# Autodesk Inventor assembly: Ball Bearing Inside Mechanics
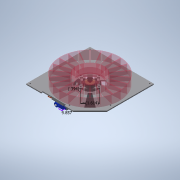
[picture p0: Inventor's stored thumbnail of the model, 180x180]
Saved by Autodesk Inventor 2022 (Build 260153000, 153)
## iProperties
Created: 2023-03-21
Part Number: Ball Bearing Inside Mechanics
Document SubType Name: Assembly
Designer: zarek
Author: zarek
## Documents named in this file (9)
- C:\Users\zarek\OneDrive\Desktop\Random New Stuff\SPB\Ball Bearing Inside Mechanics.iam
- C:\Users\zarek\OneDrive\Desktop\Random New Stuff\SPB\Capsule_Design_Revamp.ipt
- C:\Users\zarek\OneDrive\Desktop\Random New Stuff\SPB\Drop_Plate_Ball_Bearing_Cuttout.ipt
- C:\Users\zarek\OneDrive\Desktop\Random New Stuff\SPB\GrabCad Parts\Stepper 28BYJ48.ipt
- C:\Users\zarek\OneDrive\Desktop\Random New Stuff\SPB\Ball_Bearing_Holder_Assembly.iam
- C:\Users\zarek\OneDrive\Desktop\Random New Stuff\SPB\Ball_Bearing_Mock_8_22_7mm.ipt
- C:\Users\zarek\OneDrive\Desktop\Random New Stuff\SPB\Servo Holder.ipt
- C:\Users\zarek\OneDrive\Desktop\Random New Stuff\SPB\GrabCad Parts\Servo HXT900 Micro.ipt
- C:\Users\zarek\OneDrive\Desktop\Random New Stuff\SPB\Motor_Holder - Copy.ipt
## Components (8 placed, 8 different names)
1. Capsule_Design_Revamp:1 — Rigid:1
2. Stepper 28BYJ48:1 — Rotational:3
3. Ball_Bearing_Holder_Assembly:1 [sub-assembly] — Rotational:3, Rigid:1
4. Drop_Plate_Ball_Bearing_Cuttout:1 — Rigid:2, Rotational:6
5. Ball_Bearing_Mock_8_22_7mm:1
6. Servo Holder:1 — Rigid:2, Rotational:5
7. Servo HXT900 Micro:1 — Rotational:5
8. Motor_Holder - Copy:1 — Rotational:6
## Relationships (5: RevoluteJoint 3, WeldJoint 2)
- Rotational:3 [RevoluteJoint] (0.1 mm): Stepper 28BYJ48:1 ↔ Ball_Bearing_Holder_Assembly:1
- Rigid:1 [WeldJoint]: Capsule_Design_Revamp:1 ↔ Ball_Bearing_Holder_Assembly:1
- Rigid:2 [WeldJoint]: Drop_Plate_Ball_Bearing_Cuttout:1 ↔ Servo Holder:1
- Rotational:5 [RevoluteJoint]: Servo Holder:1 ↔ Servo HXT900 Micro:1
- Rotational:6 [RevoluteJoint]: Drop_Plate_Ball_Bearing_Cuttout:1 ↔ Motor_Holder - Copy:1
